# Autodesk Inventor assembly: 000ASS_Bo_banh_xe_03
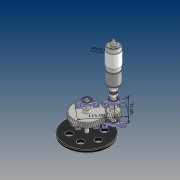
[picture p0: Inventor's stored thumbnail of the model, 180x180]
Saved by Autodesk Inventor 2021 (Build 250183000, 183)
## iProperties
Created: 2024-03-11
Part Number: 000ASS_Bo_banh_xe_03
Document SubType Name: Assembly
Designer: Admin
Author: Admin
## Documents named in this file (9)
- C:\Users\Admin\Desktop\DO_AN_TOT_NGHIEP_2024\Mechanical\Design_in_3D\Version_1\000ASS_Bo_banh_xe_03.iam
- C:\Users\Admin\Desktop\DO_AN_TOT_NGHIEP_2024\Mechanical\Design_in_3D\Library\kp08-baering-with-housing-1.snapshot.4\KP08.iam
- C:\Users\Admin\Desktop\DO_AN_TOT_NGHIEP_2024\Mechanical\Design_in_3D\Library\planetary-gear-dc-motor-2.snapshot.1\Planetary Gear DC Motor\Planatary motor v1.ipt
- C:\Users\Admin\Desktop\DO_AN_TOT_NGHIEP_2024\Mechanical\Design_in_3D\Library\kh-p-n-i-m-m-2.snapshot.1\khop-noi-mem.ipt
- C:\Users\Admin\Desktop\DO_AN_TOT_NGHIEP_2024\Mechanical\Design_in_3D\Library\Banh_rang\Banh_rang_bi_dan_02.ipt
- C:\Users\Admin\Desktop\DO_AN_TOT_NGHIEP_2024\Mechanical\Design_in_3D\Library\Banh_rang\Banh_rang_dan_02.ipt
- C:\Users\Admin\Desktop\DO_AN_TOT_NGHIEP_2024\Mechanical\Design_in_3D\Version_1\02_Truc_02.ipt
- C:\Users\Admin\Desktop\DO_AN_TOT_NGHIEP_2024\Mechanical\Design_in_3D\Version_1\05_Banh_xe.ipt
- C:\Users\Admin\Desktop\DO_AN_TOT_NGHIEP_2024\Mechanical\Design_in_3D\Version_1\01_Truc_02.ipt
## Components (11 placed, 8 different names)
1. KP08:1 [sub-assembly] — Flush:1, Flush:6, Mate:17, Mate:32
2. KP08:2 [sub-assembly] — Flush:1, Flush:4, Flush:5, Flush:14, Mate:27
3. Planatary motor v1:1 — Mate:5
4. khop-noi-mem:1 — Mate:5, Mate:17, Mate:29
5. KP08:3 [sub-assembly] — Flush:4, Flush:5, Flush:10, Mate:18, Mate:28
6. KP08:4 [sub-assembly] — Flush:6, Flush:10, Mate:19, Mate:20, Flush:11, Mate:21
7. Spur Gear2:1 — Mate:18, Mate:19, Mate:21, Flush:12, Mate:28
8. Spur Gear1:1 — Flush:12, Mate:26
9. 02_Truc_02:1 — Mate:20, Flush:11, Mate:25, Flush:13, Mate:30
10. 05_Banh_xe:1 — Mate:25, Flush:13
11. 01_Truc_02:1 — Mate:26, Flush:14, Mate:27, Mate:29, Mate:30, Mate:32
## Relationships (22: Mate 13, Flush 9)
- Flush:1: KP08:1 ↔ KP08:2
- Mate:5: Planatary motor v1:1 ↔ khop-noi-mem:1
- Flush:4: KP08:2 ↔ KP08:3
- Flush:5: KP08:2 ↔ KP08:3
- Flush:6: KP08:1 ↔ KP08:4
- Flush:10: KP08:3 ↔ KP08:4
- Mate:17 (5 mm): KP08:1 ↔ khop-noi-mem:1
- Mate:18: KP08:3 ↔ Spur Gear2:1
- Mate:19: KP08:4 ↔ Spur Gear2:1
- Mate:20: KP08:4 ↔ 02_Truc_02:1
- Flush:11: KP08:4 ↔ 02_Truc_02:1
- Mate:21 (10 mm): KP08:4 ↔ Spur Gear2:1
- Flush:12: Spur Gear2:1 ↔ Spur Gear1:1
- Mate:25: 02_Truc_02:1 ↔ 05_Banh_xe:1
- Flush:13: 02_Truc_02:1 ↔ 05_Banh_xe:1
- Mate:26: Spur Gear1:1 ↔ 01_Truc_02:1
- Flush:14: KP08:2 ↔ 01_Truc_02:1
- Mate:27: KP08:2 ↔ 01_Truc_02:1
- Mate:28 (10 mm): KP08:3 ↔ Spur Gear2:1
- Mate:29: khop-noi-mem:1 ↔ 01_Truc_02:1
- Mate:30 (60 mm): 02_Truc_02:1 ↔ 01_Truc_02:1
- Mate:32: KP08:1 ↔ 01_Truc_02:1
